# Autodesk Inventor assembly: RobotSpine
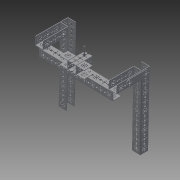
[picture p0: Inventor's stored thumbnail of the model, 180x180]
Saved by Autodesk Inventor 2015 (Build 190159000, 159)
## iProperties
Created: 2015-01-31
Part Number: RobotSpine
Document SubType Name: Assembly
Designer: sauhaarda
Author: sauhaarda
## Documents named in this file (8)
- C:\Users\Bhaskar\Desktop\RoboCAD\CAD\RobotSpine.iam
- C:\Users\Bhaskar\Desktop\RoboCAD\CAD\Imported Components\288mm Channel\Assembly3.iam
- C:\Users\Bhaskar\Desktop\RoboCAD\CAD\Imported Components\Flat Bracket\Assembly4.iam
- C:\Users\Bhaskar\Desktop\RoboCAD\CAD\Imported Components\96 mm Channel\Assembly5.iam
- C:\Users\Bhaskar\Desktop\RoboCAD\CAD\Imported Components\288mm Channel\Assembly7.iam
- C:\Users\Bhaskar\Desktop\RoboCAD\CAD\Imported Components\288mm Channel\Assembly8.iam
- C:\Users\Bhaskar\Desktop\RoboCAD\CAD\Imported Components\32mm Channel\Assembly10.iam
- C:\Users\Bhaskar\Desktop\RoboCAD\CAD\Imported Components\wormgearbox\Assembly1.iam
## Components (10 placed, 7 different names)
1. Assembly3:2 [sub-assembly] — Insert:1, Angle:1
2. Assembly4:1 [sub-assembly] — Insert:1, Angle:1, Insert:2, Angle:2
3. Assembly5:1 [sub-assembly] — Insert:2, Angle:2, Insert:6, Angle:8
4. Assembly5:2 [sub-assembly] — Insert:4, Angle:5, Insert:7, Angle:7
5. Assembly4:2 [sub-assembly] — Insert:4, Insert:5, Angle:3, Angle:5, Angle:6
6. Assembly8:1 [sub-assembly] — Insert:5, Angle:3, Angle:6
7. Assembly7:1 [sub-assembly] — Insert:6, Insert:7, Angle:7, Angle:8, Angle:9, Insert:10
8. Assembly10:1 [sub-assembly] — Angle:9, Insert:8, Angle:10
9. Assembly1:1 [sub-assembly] — Insert:8, Angle:10, Insert:9, Angle:11, Insert:10
10. Assembly10:2 [sub-assembly] — Insert:9, Angle:11
## Relationships (19: Angle 10, Insert 9)
- Insert:1: Assembly3:2 ↔ Assembly4:1
- Angle:1 (0 deg): Assembly3:2 ↔ Assembly4:1
- Insert:2: Assembly4:1 ↔ Assembly5:1
- Angle:2 (0 deg): Assembly4:1 ↔ Assembly5:1
- Insert:4: Assembly5:2 ↔ Assembly4:2
- Insert:5: Assembly4:2 ↔ Assembly8:1
- Angle:3 (0 deg): Assembly4:2 ↔ Assembly8:1
- Angle:5 (0 deg): Assembly5:2 ↔ Assembly4:2
- Angle:6 (0 deg): Assembly4:2 ↔ Assembly8:1
- Insert:6: Assembly5:1 ↔ Assembly7:1
- Insert:7: Assembly5:2 ↔ Assembly7:1
- Angle:7 (0 deg): Assembly5:2 ↔ Assembly7:1
- Angle:8 (0 deg): Assembly5:1 ↔ Assembly7:1
- Angle:9 (0 deg): Assembly7:1 ↔ Assembly10:1
- Insert:8: Assembly10:1 ↔ Assembly1:1
- Angle:10 (0 deg): Assembly10:1 ↔ Assembly1:1
- Insert:9: Assembly1:1 ↔ Assembly10:2
- Angle:11 (0 deg): Assembly1:1 ↔ Assembly10:2
- Insert:10: Assembly7:1 ↔ Assembly1:1
